# Autodesk Inventor assembly: DroneStructure
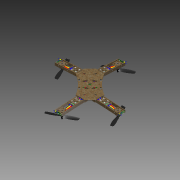
[picture p0: Inventor's stored thumbnail of the model, 180x180]
Saved by Autodesk Inventor 2012 (Build 160160000, 160)
## iProperties
Created: 2014-07-08
Part Number: DroneStructure
Document SubType Name: Assembly
Designer: Laurent
Author: Laurent
## Documents named in this file (13)
- D:\Dropbox\Courses\GP\Inventor\dronestructure\DroneStructure.iam
- D:\Dropbox\Courses\GP\Inventor\dronestructure\Centerplate.ipt
- D:\Dropbox\Courses\GP\Inventor\dronestructure\LongMiddleStructure.ipt
- D:\Dropbox\Courses\GP\Inventor\dronestructure\electronics\powerswitch\PowerSwitchBoardAssembly.iam
- D:\Dropbox\Courses\GP\Inventor\dronestructure\ShortMiddleStructure-ESCholes.ipt
- D:\Dropbox\Courses\GP\Inventor\dronestructure\LeftArm.iam
- D:\Dropbox\Courses\GP\Inventor\dronestructure\RightArm.iam
- D:\Dropbox\Courses\GP\Inventor\dronestructure\FrontLabel.ipt
- D:\Dropbox\Courses\GP\Inventor\dronestructure\BackLabel.ipt
- D:\Dropbox\Courses\GP\Inventor\dronestructure\cables\DroneStructure.FrontLeftESC.iam
- D:\Dropbox\Courses\GP\Inventor\dronestructure\cables\DroneStructure.FrontRightESC.iam
- D:\Dropbox\Courses\GP\Inventor\dronestructure\cables\DroneStructure.BackLeftESC.iam
- D:\Dropbox\Courses\GP\Inventor\dronestructure\cables\DroneStructure.BackRightESC.iam
## Components (16 placed, 16 different names)
1. FrameBase — Mate:13, Mate:14, Mate:73, Mate:74, Mate:75, Mate:87, Mate:89, Mate:90, Mate:92, Mate:93, Mate:94, Mate:95, Mate:96, Mate:106, Mate:107, Mate:108, Mate:109, Mate:110, Mate:111, Mate:112, Mate:113, Mate:114, Mate:115, Mate:116, Mate:117, Mate:118, Flush:1, Flush:3, Mate:119
2. LongMiddleSupportRight — Mate:13, Mate:14, Mate:88, Mate:91, Mate:96
3. LongMiddleSupportLeft — Mate:93, Mate:94, Mate:95
4. PowerSwitchBoard [sub-assembly] — Mate:73, Mate:74, Mate:75
5. ShortMiddleSupportBack — Mate:90, Mate:91, Mate:92
6. ShortMiddleSupportFront — Mate:87, Mate:88, Mate:89
7. FrontLeftArm [sub-assembly] — Mate:106, Mate:107, Mate:108
8. BackRightArm [sub-assembly] — Mate:109, Mate:110, Mate:111
9. FrontRightArm [sub-assembly] — Mate:112, Mate:113, Mate:114
10. BackLeftArm [sub-assembly] — Mate:115, Mate:116, Mate:117
11. FrontLabel — Mate:118, Flush:2
12. BackLabel — Mate:119, Flush:4
13. FrontLeftESC [sub-assembly]
14. FrontRightESC [sub-assembly]
15. BackLeftESC [sub-assembly]
16. BackRightESC [sub-assembly]
## Relationships (33: Mate 29, Flush 4)
- Mate:13: FrameBase ↔ LongMiddleSupportRight
- Mate:14: FrameBase ↔ LongMiddleSupportRight
- Mate:73: FrameBase ↔ PowerSwitchBoard
- Mate:74: FrameBase ↔ PowerSwitchBoard
- Mate:75: FrameBase ↔ PowerSwitchBoard
- Mate:87: FrameBase ↔ ShortMiddleSupportFront
- Mate:88: LongMiddleSupportRight ↔ ShortMiddleSupportFront
- Mate:89: FrameBase ↔ ShortMiddleSupportFront
- Mate:90: FrameBase ↔ ShortMiddleSupportBack
- Mate:91: LongMiddleSupportRight ↔ ShortMiddleSupportBack
- Mate:92: FrameBase ↔ ShortMiddleSupportBack
- Mate:93: FrameBase ↔ LongMiddleSupportLeft
- Mate:94: FrameBase ↔ LongMiddleSupportLeft
- Mate:95: FrameBase ↔ LongMiddleSupportLeft
- Mate:96: FrameBase ↔ LongMiddleSupportRight
- Mate:106: FrameBase ↔ FrontLeftArm
- Mate:107: FrameBase ↔ FrontLeftArm
- Mate:108: FrameBase ↔ FrontLeftArm
- Mate:109: FrameBase ↔ BackRightArm
- Mate:110: FrameBase ↔ BackRightArm
- Mate:111: FrameBase ↔ BackRightArm
- Mate:112: FrameBase ↔ FrontRightArm
- Mate:113: FrameBase ↔ FrontRightArm
- Mate:114: FrameBase ↔ FrontRightArm
- Mate:115: FrameBase ↔ BackLeftArm
- Mate:116: FrameBase ↔ BackLeftArm
- Mate:117: FrameBase ↔ BackLeftArm
- Mate:118: FrameBase ↔ FrontLabel
- Flush:1 (-5 mm): FrameBase
- Flush:2: FrontLabel
- Flush:3 (-5 mm): FrameBase
- Mate:119: FrameBase ↔ BackLabel
- Flush:4: BackLabel
